# Autodesk Inventor assembly: SHANK2
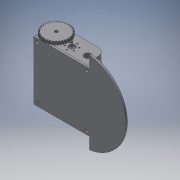
[picture p0: Inventor's stored thumbnail of the model, 180x180]
Saved by Autodesk Inventor 2019 (Build 230136000, 136)
## iProperties
Created: 2017-05-03
Part Number: SHANK2
Document SubType Name: Assembly
Designer: ANDRES
Author: ANDRES
## Documents named in this file (7)
- C:\Users\Andres\Documents\GitHub\Shank2.0\Variados\Diseño Mecanico\SHANK2.iam
- C:\Users\Andres\Documents\GitHub\Shank2.0\Variados\Diseño Mecanico\PCB_Final.ipt
- C:\Users\Andres\Documents\GitHub\Shank2.0\Variados\Diseño Mecanico\Base_Motor_acrilico_15.ipt
- C:\Users\Andres\Documents\GitHub\Shank2.0\Variados\Diseño Mecanico\Motor_Final.ipt
- C:\Users\Andres\Documents\GitHub\Shank2.0\Variados\Diseño Mecanico\Tornillo.ipt
- C:\Users\Andres\Documents\GitHub\Shank2.0\Variados\Diseño Mecanico\Spoiler.ipt
- C:\Users\Andres\Documents\GitHub\Shank2.0\Variados\Diseño Mecanico\Engranajes\Engranajes GRANDE final 2017.ipt
## Components (8 placed, 6 different names)
1. PCB_Final:1 — Mate:1, Mate:2, Mate:3, Flush:1, Mate:5, Flush:2, Mate:8
2. Base_Motor_acrilico_15:1 — Mate:2, Flush:2, Mate:8, Flush:3, Cylindrical:3
3. Base_Motor_acrilico_15:2 — Mate:3, Flush:1, Mate:5, Cylindrical:1, Mate:7, Cylindrical:4
4. Motor_Final:1 — Cylindrical:1, Mate:6, Cylindrical:2, Mate:7
5. Motor_Final:2 — Mate:6, Cylindrical:2
6. Tornillo:1 — Flush:3, Cylindrical:3
7. Spoiler:1
8. Engranajes GRANDE final 2017:1 — Cylindrical:4
## Relationships (14: Mate 7, CylindricalJoint 4, Flush 3)
- Mate:1: PCB_Final:1
- Mate:2: PCB_Final:1 ↔ Base_Motor_acrilico_15:1
- Mate:3: PCB_Final:1 ↔ Base_Motor_acrilico_15:2
- Flush:1: PCB_Final:1 ↔ Base_Motor_acrilico_15:2
- Mate:5: PCB_Final:1 ↔ Base_Motor_acrilico_15:2
- Cylindrical:1: Base_Motor_acrilico_15:2 ↔ Motor_Final:1
- Mate:6: Motor_Final:1 ↔ Motor_Final:2
- Cylindrical:2: Motor_Final:1 ↔ Motor_Final:2
- Mate:7: Base_Motor_acrilico_15:2 ↔ Motor_Final:1
- Flush:2: PCB_Final:1 ↔ Base_Motor_acrilico_15:1
- Mate:8: PCB_Final:1 ↔ Base_Motor_acrilico_15:1
- Flush:3: Base_Motor_acrilico_15:1 ↔ Tornillo:1
- Cylindrical:3: Base_Motor_acrilico_15:1 ↔ Tornillo:1
- Cylindrical:4: Base_Motor_acrilico_15:2 ↔ Engranajes GRANDE final 2017:1
